# Autodesk Inventor assembly: MARCO SP40-01 2100X800
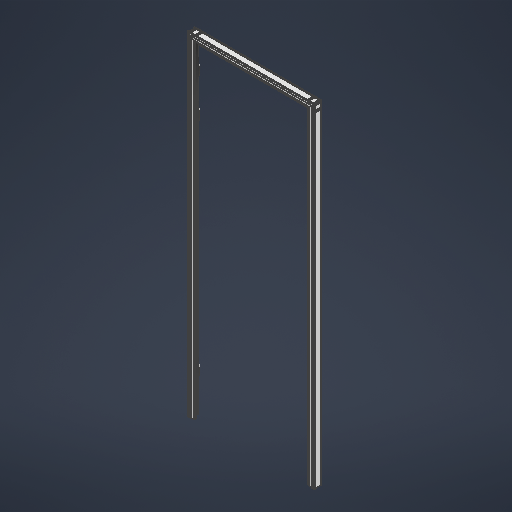
[picture p0: Inventor's stored thumbnail of the model, 512x512]
Saved by Autodesk Inventor 2025 (Build 290162000, 162)
## iProperties
Created: 2026-02-12
Part Number: MARCO SP40-01 2100X800
Document SubType Name: Assembly
Designer: Frank
Author: Frank
## Documents named in this file (12)
- C:\Users\rolan\OneDrive\Documentos\Inventor\Projects\CARPINTERIA ALUMINIO\PUERTAS Y VENTANAS\PUERTAS\MARCOS\ENSAMBLES\MARCO SP40-01 2100x800.iam
- C:\Users\rolan\OneDrive\Documentos\Inventor\Projects\CARPINTERIA ALUMINIO\PUERTAS Y VENTANAS\PUERTAS\MARCOS\PIEZAS\MARCO SP40-01 2100x800\SP40-01 MARCO BATIENTE - PAÑO FIJO 800 mm.ipt
- C:\Users\rolan\OneDrive\Documentos\Inventor\Projects\CARPINTERIA ALUMINIO\PUERTAS Y VENTANAS\PUERTAS\MARCOS\PIEZAS\MARCO SP40-01 2100x800\SP40-02 JUNTA INT 727.ipt
- C:\Users\rolan\OneDrive\Documentos\Inventor\Projects\CARPINTERIA ALUMINIO\PUERTAS Y VENTANAS\VENTANAS\MARCOS\PIEZAS\MARCO CORREDERA SP40-09 EXT 1400x1200\BRA-13 ESCUADRA UNIÓN 45 37 mm.ipt
- C:\Users\rolan\OneDrive\Documentos\Inventor\Projects\CARPINTERIA ALUMINIO\PUERTAS Y VENTANAS\PUERTAS\MARCOS\PIEZAS\MARCO SP40-01 2100x800\SP40-01 MARCO BATIENTE - PAÑO FIJO 2100 mm.ipt
- C:\Users\rolan\OneDrive\Documentos\Inventor\Projects\CARPINTERIA ALUMINIO\PUERTAS Y VENTANAS\PUERTAS\MARCOS\PIEZAS\MARCO SP40-01 2100x800\SP40-02 JUNTA INT 2063.ipt
- C:\Users\rolan\OneDrive\Documentos\Inventor\Projects\CARPINTERIA ALUMINIO\PUERTAS Y VENTANAS\PUERTAS\MARCOS\PIEZAS\MARCO SP40-01 2100x800\SP40-01 MARCO BATIENTE - PAÑO FIJO 2100 mm_MIR.ipt
- C:\Users\rolan\OneDrive\Documentos\Inventor\Projects\CARPINTERIA ALUMINIO\PUERTAS Y VENTANAS\PUERTAS\MARCOS\PIEZAS\MARCO SP40-01 2100x800\SP40-02 JUNTA INT 2063_MIR.ipt
- C:\Users\rolan\OneDrive\Documentos\Inventor\Projects\CARPINTERIA ALUMINIO\PUERTAS Y VENTANAS\PUERTAS\MARCOS\PIEZAS\MARCO SP40-01 2100x800\BRA-13 ESCUADRA UNIÓN 45 14 mm_MIR.ipt
- C:\Users\rolan\OneDrive\Documentos\Inventor\Projects\CARPINTERIA ALUMINIO\PUERTAS Y VENTANAS\ACCESORIOS\BISAGRAS\ENSAMBLES\HIN-61 BISAGRA (P1 MARCO-PASADOR).iam
- HIN-61 BISAGRA (P1 MARCO-PASADOR).iam
- C:\Users\rolan\Documents\Inventor\Content Center Files\R2025\es-ES\ISO 10642(2)\ISO 10642  - M6  x  8.ipt
## Components (12 placed, 10 different names)
1. SP40-01 MARCO BATIENTE - PAÑO FIJO 800 mm:1 — Coincidencia:1, Coincidencia:2, Coincidencia:3, Coincidencia:6, Coincidencia:7, Coincidencia:8, Coincidencia:12, Coincidencia:13, Coincidencia:19, Coincidencia:20, Coincidencia:21, Coincidencia:22, Coincidencia:23, Nivelación:1
2. SP40-02 JUNTA INT 727:1 — Coincidencia:1, Coincidencia:2, Coincidencia:3
3. SP40-01 MARCO BATIENTE - PAÑO FIJO 2100 mm:1 — Coincidencia:6, Coincidencia:7, Coincidencia:8, Coincidencia:9, Coincidencia:10, Coincidencia:11, Coincidencia:14, Coincidencia:24, Coincidencia:25, Coincidencia:26, Coincidencia:27, Coincidencia:28, Nivelación:2
4. SP40-02 JUNTA INT 2063:1 — Coincidencia:9, Coincidencia:10, Coincidencia:11
5. BRA-13 ESCUADRA UNIÓN 45 37 mm:1 — Coincidencia:12, Coincidencia:13, Coincidencia:14
6. SP40-01 MARCO BATIENTE - PAÑO FIJO 2100 mm_MIR:1 — Coincidencia:15, Coincidencia:16, Coincidencia:17, Coincidencia:18, Coincidencia:20, Coincidencia:22, Coincidencia:29
7. SP40-02 JUNTA INT 2063_MIR:1 — Coincidencia:15, Coincidencia:16, Coincidencia:17
8. BRA-13 ESCUADRA UNIÓN 45 14 mm_MIR:1 — Coincidencia:18, Coincidencia:19, Coincidencia:21
9. HIN-61 BISAGRA (P1 MARCO-PASADOR):3 [sub-assembly] — Coincidencia:27, Coincidencia:28, Nivelación:2
10. DIN EN ISO 10642 M6  x  8:1 — Coincidencia:29
11. HIN-61 BISAGRA (P1 MARCO-PASADOR):1 [sub-assembly] — Coincidencia:25, Coincidencia:26, Nivelación:1
12. HIN-61 BISAGRA (P1 MARCO-PASADOR):2 [sub-assembly]
## Component patterns: (2 elements, first: HIN-61 BISAGRA (P1 MARCO-PASADOR):1)
## Relationships (29: Mate 27, Flush 2)
- Coincidencia:1 [Mate]: SP40-01 MARCO BATIENTE - PAÑO FIJO 800 mm:1 ↔ SP40-02 JUNTA INT 727:1
- Coincidencia:2 [Mate]: SP40-01 MARCO BATIENTE - PAÑO FIJO 800 mm:1 ↔ SP40-02 JUNTA INT 727:1
- Coincidencia:3 [Mate]: SP40-01 MARCO BATIENTE - PAÑO FIJO 800 mm:1 ↔ SP40-02 JUNTA INT 727:1
- Coincidencia:6 [Mate]: SP40-01 MARCO BATIENTE - PAÑO FIJO 800 mm:1 ↔ SP40-01 MARCO BATIENTE - PAÑO FIJO 2100 mm:1
- Coincidencia:7 [Mate]: SP40-01 MARCO BATIENTE - PAÑO FIJO 800 mm:1 ↔ SP40-01 MARCO BATIENTE - PAÑO FIJO 2100 mm:1
- Coincidencia:8 [Mate]: SP40-01 MARCO BATIENTE - PAÑO FIJO 800 mm:1 ↔ SP40-01 MARCO BATIENTE - PAÑO FIJO 2100 mm:1
- Coincidencia:9 [Mate]: SP40-01 MARCO BATIENTE - PAÑO FIJO 2100 mm:1 ↔ SP40-02 JUNTA INT 2063:1
- Coincidencia:10 [Mate]: SP40-01 MARCO BATIENTE - PAÑO FIJO 2100 mm:1 ↔ SP40-02 JUNTA INT 2063:1
- Coincidencia:11 [Mate]: SP40-01 MARCO BATIENTE - PAÑO FIJO 2100 mm:1 ↔ SP40-02 JUNTA INT 2063:1
- Coincidencia:12 [Mate]: SP40-01 MARCO BATIENTE - PAÑO FIJO 800 mm:1 ↔ BRA-13 ESCUADRA UNIÓN 45 37 mm:1
- Coincidencia:13 [Mate] (1 mm): SP40-01 MARCO BATIENTE - PAÑO FIJO 800 mm:1 ↔ BRA-13 ESCUADRA UNIÓN 45 37 mm:1
- Coincidencia:14 [Mate]: SP40-01 MARCO BATIENTE - PAÑO FIJO 2100 mm:1 ↔ BRA-13 ESCUADRA UNIÓN 45 37 mm:1
- Coincidencia:15 [Mate]: SP40-01 MARCO BATIENTE - PAÑO FIJO 2100 mm_MIR:1 ↔ SP40-02 JUNTA INT 2063_MIR:1
- Coincidencia:16 [Mate]: SP40-01 MARCO BATIENTE - PAÑO FIJO 2100 mm_MIR:1 ↔ SP40-02 JUNTA INT 2063_MIR:1
- Coincidencia:17 [Mate]: SP40-01 MARCO BATIENTE - PAÑO FIJO 2100 mm_MIR:1 ↔ SP40-02 JUNTA INT 2063_MIR:1
- Coincidencia:18 [Mate]: SP40-01 MARCO BATIENTE - PAÑO FIJO 2100 mm_MIR:1 ↔ BRA-13 ESCUADRA UNIÓN 45 14 mm_MIR:1
- Coincidencia:19 [Mate]: SP40-01 MARCO BATIENTE - PAÑO FIJO 800 mm:1 ↔ BRA-13 ESCUADRA UNIÓN 45 14 mm_MIR:1
- Coincidencia:20 [Mate]: SP40-01 MARCO BATIENTE - PAÑO FIJO 800 mm:1 ↔ SP40-01 MARCO BATIENTE - PAÑO FIJO 2100 mm_MIR:1
- Coincidencia:21 [Mate] (1 mm): SP40-01 MARCO BATIENTE - PAÑO FIJO 800 mm:1 ↔ BRA-13 ESCUADRA UNIÓN 45 14 mm_MIR:1
- Coincidencia:22 [Mate]: SP40-01 MARCO BATIENTE - PAÑO FIJO 800 mm:1 ↔ SP40-01 MARCO BATIENTE - PAÑO FIJO 2100 mm_MIR:1
- Coincidencia:23 [Mate]: SP40-01 MARCO BATIENTE - PAÑO FIJO 800 mm:1
- Coincidencia:24 [Mate]: SP40-01 MARCO BATIENTE - PAÑO FIJO 2100 mm:1
- Coincidencia:25 [Mate]: SP40-01 MARCO BATIENTE - PAÑO FIJO 2100 mm:1 ↔ HIN-61 BISAGRA (P1 MARCO-PASADOR):1
- Coincidencia:26 [Mate]: SP40-01 MARCO BATIENTE - PAÑO FIJO 2100 mm:1 ↔ HIN-61 BISAGRA (P1 MARCO-PASADOR):1
- Nivelación:1 [Flush] (210 mm): SP40-01 MARCO BATIENTE - PAÑO FIJO 800 mm:1 ↔ HIN-61 BISAGRA (P1 MARCO-PASADOR):1
- Coincidencia:27 [Mate]: SP40-01 MARCO BATIENTE - PAÑO FIJO 2100 mm:1 ↔ HIN-61 BISAGRA (P1 MARCO-PASADOR):3
- Coincidencia:28 [Mate]: SP40-01 MARCO BATIENTE - PAÑO FIJO 2100 mm:1 ↔ HIN-61 BISAGRA (P1 MARCO-PASADOR):3
- Nivelación:2 [Flush] (210 mm): SP40-01 MARCO BATIENTE - PAÑO FIJO 2100 mm:1 ↔ HIN-61 BISAGRA (P1 MARCO-PASADOR):3
- Coincidencia:29 [Mate]: SP40-01 MARCO BATIENTE - PAÑO FIJO 2100 mm_MIR:1 ↔ DIN EN ISO 10642 M6  x  8:1
